# Autodesk Inventor assembly: !Structure
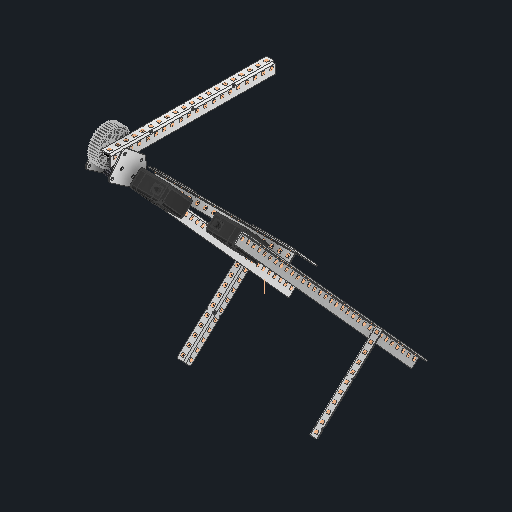
[picture p0: Inventor's stored thumbnail of the model, 512x512]
Saved by Autodesk Inventor 2025 (Build 290162000, 162)
## iProperties
Created: 2024-12-30
Part Number: !Structure
Document SubType Name: Assembly
Designer: Averey Ku
Author: Averey Ku
## Documents named in this file (13)
- D:\VEX\High Stakes\CAD\V4\Lady Brown\Structure\!Structure.iam
- D:\VEX\High Stakes\CAD\ROBOPROS-CAD-Inventor\Structure\C Channel\Aluminum 1x3x1 Half Thick Cut\Alu C Half Thick 1x3x1x32.ipt
- D:\VEX\High Stakes\CAD\ROBOPROS-CAD-Inventor\Structure\Angle\Aluminum 1x1\Alu Angle 1x1x12.ipt
- D:\VEX\High Stakes\CAD\ROBOPROS-CAD-Inventor\Structure\Angle\Aluminum 1x1\Alu Angle 1x1x11.ipt
- D:\VEX\High Stakes\CAD\V4\Lady Brown\Structure\Custom Parts\Gearbox.ipt
- D:\VEX\High Stakes\CAD\ROBOPROS-CAD-Inventor\Electronics\V5 Motor (5.5W).ipt
- D:\VEX\High Stakes\CAD\ROBOPROS-CAD-Inventor\Structure\C Channel\Aluminum 1x3x1 Half Thick Cut\Alu C Half Thick 1x3x1x17.ipt
- D:\VEX\High Stakes\CAD\V4\Lady Brown\Structure\Custom Parts\Triangle Gusset.ipt
- D:\VEX\High Stakes\CAD\ROBOPROS-CAD-Inventor\Motion\Gears\HS Gear.iam
- D:\VEX\High Stakes\CAD\ROBOPROS-CAD-Inventor\Motion\Gears\HS Gear\HS 24T Gear, No Insert.iam
- D:\VEX\High Stakes\CAD\ROBOPROS-CAD-Inventor\Structure\C Channel\Aluminum 1x3x1 Half Thick Cut\Alu C Half Thick 1x3x1x31.ipt
- D:\VEX\High Stakes\CAD\V4\Lady Brown\Arm\Right.iam
- D:\VEX\High Stakes\CAD\ROBOPROS-CAD-Inventor\Structure\Hardware\Nut Keps.ipt
## Components (17 placed, 11 different names)
1. Alu C Half Thick 1x3x1x32:1 — Insert:2, Flush:1, Mate:13, Insert:20, Mate:16, Insert:21, Mate:17, Insert:25, Mate:22
2. Alu Angle 1x1x12:1 — Mate:2
3. Alu Angle 1x1x11:1 — Insert:2, Mate:2
4. V5 Motor (5.5W):1 — Insert:20, Mate:16
5. Alu C Half Thick 1x3x1x32:2 — Mate:6, Insert:9, Mate:7, Insert:10, Mate:10, Insert:14, Insert:17
6. Alu Angle 1x1x12:2 — Insert:9, Mate:7, Mate:8
7. Alu Angle 1x1x11:2 — Mate:8, Insert:10
8. V5 Motor (5.5W):2 — Mate:10, Insert:14
9. Alu C Half Thick 1x3x1x17:1 — Insert:17, Mate:13, Insert:18, Mate:14, Insert:19, Mate:15
10. Triangle Gusset:1 — Insert:18, Mate:14
11. Triangle Gusset:2 — Insert:19, Mate:15
12. Gearbox:1 — Insert:21, Mate:17, Insert:26
13. HS 24T Gear, No Insert:2 [sub-assembly]
14. Alu C Half Thick 1x3x1x31:1 — Insert:25, Mate:22, Mate:23, Insert:29
15. Right:1 [sub-assembly] — Insert:26, Mate:24
16. Gearbox:2 — Insert:28, Mate:23, Mate:24, Insert:29
17. Nut Keps:1 — Insert:28
## Relationships (29: Mate 14, Insert 14, Flush 1)
- [Mate]: Alu C Half Thick 1x3x1x32:1 ↔ Alu Angle 1x1x12:1
- [Insert]: Alu C Half Thick 1x3x1x32:1 ↔ Alu Angle 1x1x12:1
- Insert:2: Alu C Half Thick 1x3x1x32:1 ↔ Alu Angle 1x1x11:1
- Mate:2: Alu Angle 1x1x12:1 ↔ Alu Angle 1x1x11:1
- Flush:1 (93.6625 mm): Alu C Half Thick 1x3x1x32:1
- Mate:6 (93.6625 mm): Alu C Half Thick 1x3x1x32:2
- Insert:9: Alu C Half Thick 1x3x1x32:2 ↔ Alu Angle 1x1x12:2
- Mate:7: Alu C Half Thick 1x3x1x32:2 ↔ Alu Angle 1x1x12:2
- Mate:8: Alu Angle 1x1x12:2 ↔ Alu Angle 1x1x11:2
- Insert:10: Alu C Half Thick 1x3x1x32:2 ↔ Alu Angle 1x1x11:2
- Mate:10: Alu C Half Thick 1x3x1x32:2 ↔ V5 Motor (5.5W):2
- Insert:14: Alu C Half Thick 1x3x1x32:2 ↔ V5 Motor (5.5W):2
- Insert:17 (12.7 mm): Alu C Half Thick 1x3x1x32:2 ↔ Alu C Half Thick 1x3x1x17:1
- Mate:13: Alu C Half Thick 1x3x1x32:1 ↔ Alu C Half Thick 1x3x1x17:1
- Insert:18: Alu C Half Thick 1x3x1x17:1 ↔ Triangle Gusset:1
- Mate:14: Alu C Half Thick 1x3x1x17:1 ↔ Triangle Gusset:1
- Insert:19: Alu C Half Thick 1x3x1x17:1 ↔ Triangle Gusset:2
- Mate:15: Alu C Half Thick 1x3x1x17:1 ↔ Triangle Gusset:2
- Insert:20 (1.5875 mm): Alu C Half Thick 1x3x1x32:1 ↔ V5 Motor (5.5W):1
- Mate:16: Alu C Half Thick 1x3x1x32:1 ↔ V5 Motor (5.5W):1
- Insert:21 (1.5875 mm): Alu C Half Thick 1x3x1x32:1 ↔ Gearbox:1
- Mate:17: Alu C Half Thick 1x3x1x32:1 ↔ Gearbox:1
- Insert:25: Alu C Half Thick 1x3x1x32:1 ↔ Alu C Half Thick 1x3x1x31:1
- Mate:22: Alu C Half Thick 1x3x1x32:1 ↔ Alu C Half Thick 1x3x1x31:1
- Insert:26 (1.5875 mm): Gearbox:1 ↔ Right:1
- Insert:28: Gearbox:2 ↔ Nut Keps:1
- Mate:23: Alu C Half Thick 1x3x1x31:1 ↔ Gearbox:2
- Mate:24: Right:1 ↔ Gearbox:2
- Insert:29 (30.1625 mm): Alu C Half Thick 1x3x1x31:1 ↔ Gearbox:2
